# Autodesk Inventor assembly: Ultrasonic Sensor
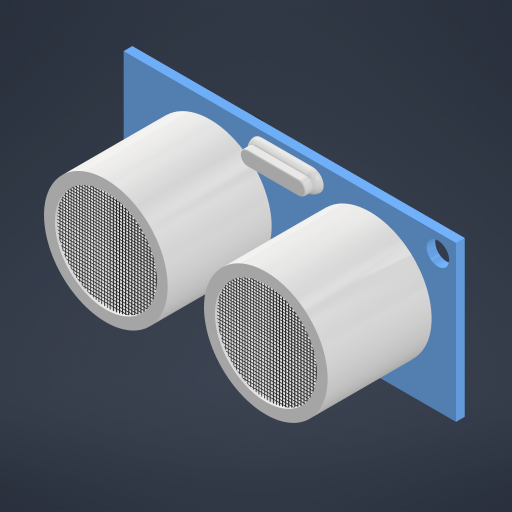
[picture p0: Inventor's stored thumbnail of the model, 512x512]
Saved by Autodesk Inventor 2024 (Build 280153000, 153)
## iProperties
Created: 2025-11-28
Part Number: Ultrasonic Sensor
Document SubType Name: Assembly
Designer: Vincent Larson
Author: Vincent Larson
## Documents named in this file (3)
- C:\Users\Vincent Larson\Downloads\Digital Ship Challenge\Digital Ship Challenge Robot\Ultrasonic sensor\Ultrasonic Sensor.iam
- C:\Users\Vincent Larson\Downloads\Digital Ship Challenge\Digital Ship Challenge Robot\Ultrasonic sensor\Ultrasonic sensor board.ipt
- C:\Users\Vincent Larson\Downloads\Digital Ship Challenge\Digital Ship Challenge Robot\Ultrasonic sensor\Ultrasonic sensor piece.ipt
## Components (3 placed, 2 different names)
1. Ultrasonic sensor board:1 — Mate:1, Mate:2
2. Ultrasonic sensor piece:1 — Mate:1
3. Ultrasonic sensor piece:2 — Mate:2
## Relationships (2: Mate 2)
- Mate:1: Ultrasonic sensor board:1 ↔ Ultrasonic sensor piece:1
- Mate:2: Ultrasonic sensor board:1 ↔ Ultrasonic sensor piece:2
